# Autodesk Inventor assembly: Z flange
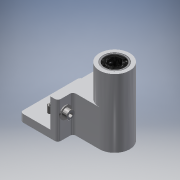
[picture p0: Inventor's stored thumbnail of the model, 180x180]
Saved by Autodesk Inventor 2018 (Build 220112000, 112)
## iProperties
Part Number: Z flange
Material: Generisch
Document SubType Name: Assembly
Designer: Till
Author: Till
## Documents named in this file (4)
- C:\Users\Till\Dropbox\Ultibox\ultibox\cad\Z flange.iam
- C:\Users\Till\Dropbox\Ultibox\ultibox\cad\flange.ipt
- C:\Users\Till\Dropbox\Ultibox\ultibox\cad\M3 x 10.ipt
- C:\Users\Till\Dropbox\Ultibox\ultibox\cad\lm8luu.ipt
## Components (6 placed, 3 different names)
1. flange:1 — Passend:2, Passend:3, Passend:4, Passend:5, Passend:6, Passend:7, Passend:8, Passend:9, Fluchtend:4
2. M3 x 10:1 — Fluchtend:2, Passend:3, Passend:4
3. M3 x 10:2 — Fluchtend:2, Passend:5
4. M3 x 10:3 — Fluchtend:3, Passend:6, Passend:7
5. M3 x 10:4 — Fluchtend:3, Passend:8
6. lm8luu:1 — Passend:9, Fluchtend:4
## Relationships (11: Mate 8, Flush 3)
- Passend:2 [Mate]: flange:1
- Fluchtend:2 [Flush]: M3 x 10:1 ↔ M3 x 10:2
- Fluchtend:3 [Flush]: M3 x 10:3 ↔ M3 x 10:4
- Passend:3 [Mate]: flange:1 ↔ M3 x 10:1
- Passend:4 [Mate]: flange:1 ↔ M3 x 10:1
- Passend:5 [Mate]: flange:1 ↔ M3 x 10:2
- Passend:6 [Mate]: flange:1 ↔ M3 x 10:3
- Passend:7 [Mate]: flange:1 ↔ M3 x 10:3
- Passend:8 [Mate]: flange:1 ↔ M3 x 10:4
- Passend:9 [Mate]: flange:1 ↔ lm8luu:1
- Fluchtend:4 [Flush]: flange:1 ↔ lm8luu:1
